# Autodesk Inventor assembly: Mid Crossbrace
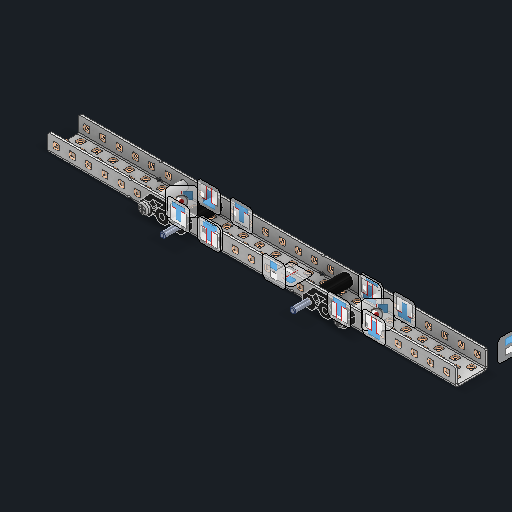
[picture p0: Inventor's stored thumbnail of the model, 512x512]
Saved by Autodesk Inventor 2025.1 (Build 291241000, 241)
## iProperties
Created: 2024-11-11
Part Number: Mid Crossbrace
Document SubType Name: Assembly
Designer: avere
Author: avere
## Documents named in this file (10)
- C:\Users\avere\VEX\High Stakes\CAD\V3\Chassis\Structure\Mid Crossbrace.iam
- C:\Users\avere\VEX\High Stakes\CAD\ROBOPROS-CAD-Inventor\Structure\C Channel\Aluminum 1x2x1\Alu C 1x2x1x25.ipt
- C:\Users\avere\VEX\High Stakes\CAD\ROBOPROS-CAD-Inventor\Motion\Shaft LS\Bearing Flat.ipt
- C:\Users\avere\VEX\High Stakes\CAD\ROBOPROS-CAD-Inventor\Motion\Spacers\Spacer Nylon .375 OD\NSpacer .375 OD x .875.ipt
- C:\Users\avere\VEX\High Stakes\CAD\ROBOPROS-CAD-Inventor\Motion\Spacers\Spacer Nylon .375 OD.ipt
- C:\Users\avere\VEX\High Stakes\CAD\ROBOPROS-CAD-Inventor\Structure\Hardware\Screw Nylon - Pan Head\NScrew Pan Head Threaded .500.ipt
- C:\Users\avere\VEX\High Stakes\CAD\ROBOPROS-CAD-Inventor\Structure\Hardware\Screw Steel - Star.ipt
- C:\Users\avere\VEX\High Stakes\CAD\ROBOPROS-CAD-Inventor\Structure\Hardware\Screw Steel - Star\SScrew Star Smooth 1.750.ipt
- C:\Users\avere\VEX\High Stakes\CAD\ROBOPROS-CAD-Inventor\Structure\Hardware\Screw Nylon - Pan Head\NScrew Pan Head Threaded .250.ipt
- C:\Users\avere\VEX\High Stakes\CAD\ROBOPROS-CAD-Inventor\Structure\Nylon Standoff Rounded\Nylon Standoff .875.ipt
## Components (13 placed, 7 different names)
1. Alu C 1x2x1x25:1 — Flush:2, Mate:2, Flush:4, Insert:18, Mate:8, Insert:19, Insert:20, Mate:9, Insert:21, Insert:26, Insert:27, Insert:29, Insert:30, Insert:32, Insert:33
2. Bearing Flat:1 — Insert:18, Mate:8, Insert:28
3. NSpacer .375 OD x .875:1 — Insert:19
4. Bearing Flat:2 — Insert:20, Mate:9, Insert:31
5. NSpacer .375 OD x .875:2 — Insert:21
6. NScrew Pan Head Threaded .500:1 — Insert:28
7. SScrew Star Smooth 1.750:1 — Insert:26
8. SScrew Star Smooth 1.750:2 — Insert:27
9. NScrew Pan Head Threaded .250:1 — Insert:29
10. Nylon Standoff .875:1 — Insert:30
11. NScrew Pan Head Threaded .500:3 — Insert:31
12. NScrew Pan Head Threaded .250:2 — Insert:33
13. Nylon Standoff .875:2 — Insert:32
## Relationships (17: Insert 12, Mate 3, Flush 2)
- Flush:2 (-158.75 mm): Alu C 1x2x1x25:1
- Mate:2 (7.9375 mm): Alu C 1x2x1x25:1
- Flush:4 (63.4238 mm): Alu C 1x2x1x25:1
- Insert:18: Alu C 1x2x1x25:1 ↔ Bearing Flat:1
- Mate:8: Alu C 1x2x1x25:1 ↔ Bearing Flat:1
- Insert:19: Alu C 1x2x1x25:1 ↔ NSpacer .375 OD x .875:1
- Insert:20: Alu C 1x2x1x25:1 ↔ Bearing Flat:2
- Mate:9: Alu C 1x2x1x25:1 ↔ Bearing Flat:2
- Insert:21: Alu C 1x2x1x25:1 ↔ NSpacer .375 OD x .875:2
- Insert:26: Alu C 1x2x1x25:1 ↔ SScrew Star Smooth 1.750:1
- Insert:27: Alu C 1x2x1x25:1 ↔ SScrew Star Smooth 1.750:2
- Insert:28: Bearing Flat:1 ↔ NScrew Pan Head Threaded .500:1
- Insert:29: Alu C 1x2x1x25:1 ↔ NScrew Pan Head Threaded .250:1
- Insert:30: Alu C 1x2x1x25:1 ↔ Nylon Standoff .875:1
- Insert:31: Bearing Flat:2 ↔ NScrew Pan Head Threaded .500:3
- Insert:32: Alu C 1x2x1x25:1 ↔ Nylon Standoff .875:2
- Insert:33: Alu C 1x2x1x25:1 ↔ NScrew Pan Head Threaded .250:2
